# Autodesk Inventor assembly: GE-12103_MIR
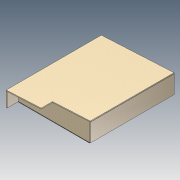
[picture p0: Inventor's stored thumbnail of the model, 180x180]
Saved by Autodesk Inventor 2012 (Build 160160000, 160)
## iProperties
Created: 2011-11-27
Part Number: GE-12103_MIR
Description: Fender, Assembly
Document SubType Name: Assembly
Designer: dfoster
Title: Fender, Assembly
Author: dfoster
## Documents named in this file (7)
- C:\Data Folder\FRC 2012 Field\Components\GE-12103_MIR.iam
- C:\Data Folder\FRC 2012 Field\Components\GE-12103-01.ipt
- C:\Data Folder\FRC 2012 Field\Components\GE-12103-02.ipt
- C:\Data Folder\FRC 2012 Field\Components\GE-12103-03.ipt
- C:\Data Folder\FRC 2012 Field\Components\GE-12103-04.ipt
- C:\Data Folder\FRC 2012 Field\Components\GE-12103-05.ipt
- C:\Data Folder\FRC 2012 Field\Components\GE-12103-06.ipt
## Components (13 placed, 6 different names)
1. GE-12103-01:1 — Mate:9, Flush:11, Flush:10, Flush:8, Flush:7, Mate:1, Mate:8, Mate:3, Flush:12, Mate:12, Flush:17, Mate:15, Flush:18, Flush:21, Flush:22, Mate:18, Mate:20
2. GE-12103-01:2 — Mate:9, Flush:11, Flush:10, Flush:6, Flush:1
3. GE-12103-01:3 — Flush:6, Flush:1, Flush:9, Mate:14, Flush:13, Mate:10, Mate:16, Flush:24
4. GE-12103-02:1 — Flush:9, Flush:8, Flush:7, Mate:1, Mate:6, Mate:5, Mate:2, Mate:7, Mate:11, Mate:17, Flush:20, Mate:17, Flush:22, Mate:18, Mate:19
5. GE-12103-03:1 — Mate:8, Mate:6, Flush:14, Flush:15
6. GE-12103-03:2 — Mate:14, Mate:5, Flush:13, Flush:19, Mate:18
7. GE-12103-03:3 — Mate:3, Mate:2, Flush:12, Mate:13, Flush:16, Flush:21, Mate:19
8. GE-12103-03:4 — Flush:14, Mate:10, Mate:7
9. GE-12103-03:5 — Flush:15, Mate:13, Mate:12, Mate:11, Mate:17
10. GE-12103-04:1 — Flush:17, Flush:16, Mate:15, Flush:23, Flush:24
11. GE-12103-05:1 — Mate:17, Flush:18, Mate:16, Flush:21, Mate:19, Mate:20, Flush:23
12. GE-12103-06:1 — Flush:20, Flush:19, Mate:18, Flush:22
13. GE-12103-06:2 — Flush:22, Flush:21, Mate:19
## Relationships (44: Flush 24, Mate 20)
- Mate:9 (-546.1 mm): GE-12103-01:1 ↔ GE-12103-01:2
- Flush:11: GE-12103-01:1 ↔ GE-12103-01:2
- Flush:10: GE-12103-01:1 ↔ GE-12103-01:2
- Flush:6: GE-12103-01:2 ↔ GE-12103-01:3
- Flush:1: GE-12103-01:2 ↔ GE-12103-01:3
- Flush:9 [Mate] (-152.4 mm): GE-12103-01:3 ↔ GE-12103-02:1
- Flush:8: GE-12103-01:1 ↔ GE-12103-02:1
- Flush:7 [Mate]: GE-12103-01:1 ↔ GE-12103-02:1
- Mate:1 [Flush]: GE-12103-01:1 ↔ GE-12103-02:1
- Mate:8 (-266.7 mm): GE-12103-01:1 ↔ GE-12103-03:1
- Mate:6 [Flush]: GE-12103-02:1 ↔ GE-12103-03:1
- Mate:14 [Flush]: GE-12103-01:3 ↔ GE-12103-03:2
- Mate:5 [Flush]: GE-12103-02:1 ↔ GE-12103-03:2
- Flush:13 [Mate]: GE-12103-01:3 ↔ GE-12103-03:2
- Mate:3 [Flush]: GE-12103-01:1 ↔ GE-12103-03:3
- Mate:2 [Flush]: GE-12103-02:1 ↔ GE-12103-03:3
- Flush:12 [Mate]: GE-12103-01:1 ↔ GE-12103-03:3
- Flush:14: GE-12103-03:1 ↔ GE-12103-03:4
- Mate:10 (-266.7 mm): GE-12103-01:3 ↔ GE-12103-03:4
- Mate:7 [Flush]: GE-12103-02:1 ↔ GE-12103-03:4
- Flush:15 [Mate]: GE-12103-03:1 ↔ GE-12103-03:5
- Mate:13 (190.5 mm): GE-12103-03:3 ↔ GE-12103-03:5
- Mate:12 [Flush]: GE-12103-01:1 ↔ GE-12103-03:5
- Mate:11 [Flush]: GE-12103-02:1 ↔ GE-12103-03:5
- Flush:17 [Mate]: GE-12103-01:1 ↔ GE-12103-04:1
- Flush:16 [Mate]: GE-12103-03:3 ↔ GE-12103-04:1
- Mate:15 [Flush]: GE-12103-01:1 ↔ GE-12103-04:1
- Mate:17: GE-12103-02:1 ↔ GE-12103-05:1
- Flush:18 [Mate]: GE-12103-01:1 ↔ GE-12103-05:1
- Mate:16 [Flush]: GE-12103-01:3 ↔ GE-12103-05:1
- Flush:20 [Mate] (6.35 mm): GE-12103-02:1 ↔ GE-12103-06:1
- Flush:19 [Mate]: GE-12103-03:2 ↔ GE-12103-06:1
- Mate:18 [Flush]: GE-12103-03:2 ↔ GE-12103-06:1
- Flush:22: GE-12103-06:1 ↔ GE-12103-06:2
- Flush:21 [Mate]: GE-12103-03:3 ↔ GE-12103-06:2
- Mate:19 [Flush]: GE-12103-03:3 ↔ GE-12103-06:2
- Flush:21: GE-12103-01:1 ↔ GE-12103-05:1
- Mate:17: GE-12103-02:1 ↔ GE-12103-03:5
- Flush:22: GE-12103-01:1 ↔ GE-12103-02:1
- Mate:18: GE-12103-01:1 ↔ GE-12103-02:1
- Mate:19: GE-12103-02:1 ↔ GE-12103-05:1
- Mate:20: GE-12103-01:1 ↔ GE-12103-05:1
- Flush:23: GE-12103-04:1 ↔ GE-12103-05:1
- Flush:24: GE-12103-01:3 ↔ GE-12103-04:1
